# Autodesk Inventor assembly: каретка
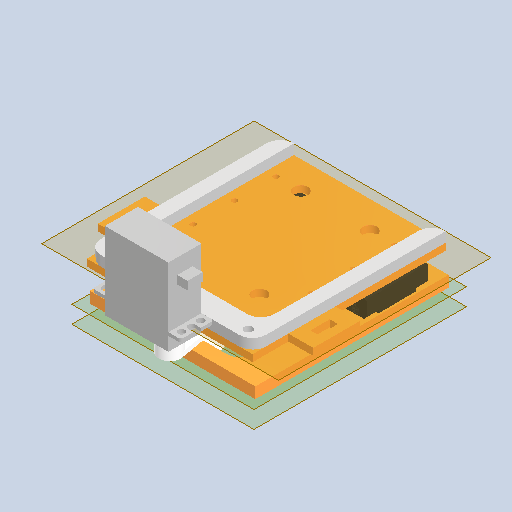
[picture p0: Inventor's stored thumbnail of the model, 512x512]
Saved by Autodesk Inventor 2024.2 (Build 282272000, 272)
## iProperties
Created: 1900-01-01
Part Number: каретка
Description: NONE
Document SubType Name: Assembly
Designer: Zakhar
Author: Zakhar
Revision Number: ANYUNSPECIFIED
## Documents named in this file (11)
- C:\Users\Service\Documents\Artist\3D\каретка.iam
- C:\Users\Service\Documents\Artist\3D\стл\Сборка плоттер\Сервопривод.ipt
- C:\Users\Service\Documents\Artist\3D\стл\Сборка плоттер\Пластина.ipt
- C:\Users\Service\Documents\Artist\3D\стл\Сборка плоттер\MGN7 rail_100 mm.ipt
- C:\Users\Service\Documents\Artist\3D\стл\Сборка плоттер\MGN7C_MGN7C.ipt
- C:\Users\Service\Documents\Artist\3D\стл\Сборка плоттер\Каретка-втулки.ipt
- C:\Users\Service\Documents\Artist\3D\стл\Сборка плоттер\Деталь.ipt
- C:\Users\Service\Documents\Artist\3D\стл\Сборка плоттер\Деталь_1.ipt
- C:\Users\Service\Documents\Artist\3D\соединялка.ipt
- C:\Users\Service\Documents\Artist\3D\стл\маркер крепление маркера.ipt
- C:\Users\Service\Documents\Artist\3D\стл\маркеркрепление маркера.ipt
## Components (11 placed, 3 different names)
1. ANY
2. ANY:5 — Заподлицо:3, Заподлицо:4
3. ANY:6
4. ANY:7
5. ANY:8
6. ANY:9
7. ANY:13 — Заподлицо:1, Заподлицо:2
8. ANY:14
9. ANY:15
10. соединялка:1 — Заподлицо:1, Заподлицо:2
11. маркер крепление маркера:1 — Заподлицо:3, Заподлицо:4
## Relationships (4: Flush 4)
- Заподлицо:1 [Flush]: ANY:13 ↔ соединялка:1
- Заподлицо:2 [Flush]: ANY:13 ↔ соединялка:1
- Заподлицо:3 [Flush]: ANY:5 ↔ маркер крепление маркера:1
- Заподлицо:4 [Flush]: ANY:5 ↔ маркер крепление маркера:1
